# Autodesk Inventor assembly: assembly1
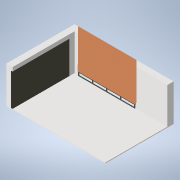
[picture p0: Inventor's stored thumbnail of the model, 180x180]
Saved by Autodesk Inventor 2021 (Build 250183000, 183)
## iProperties
Created: 2023-12-08
Part Number: assembly1
Document SubType Name: Assembly
Designer: assman
Author: assman
## Documents named in this file (5)
- D:\3DPrinting\3DModels\roco\assembly1.iam
- D:\3DPrinting\3DModels\roco\static.ipt
- D:\3DPrinting\3DModels\roco\structure.ipt
- D:\3DPrinting\3DModels\roco\zocalo_superior.ipt
- D:\3DPrinting\3DModels\roco\madera.ipt
## Components (6 placed, 4 different names)
1. static:1 — Mate:1, Mate:2, Mate:3
2. structure:1 — Mate:1, Mate:2, Mate:3, Rotational:1
3. zocalo_superior:1 — Rotational:1, Mate:4, Mate:5, Mate:6, Mate:8, Mate:9, Mate:11
4. madera:1 — Mate:4, Mate:5, Mate:7
5. madera:2 — Mate:6, Mate:7, Mate:8, Mate:10
6. madera:3 — Mate:9, Mate:10, Mate:11
## Relationships (12: Mate 11, RevoluteJoint 1)
- Mate:1 (270 mm): static:1 ↔ structure:1
- Mate:2: static:1 ↔ structure:1
- Mate:3: static:1 ↔ structure:1
- Rotational:1 [RevoluteJoint]: structure:1 ↔ zocalo_superior:1
- Mate:4: zocalo_superior:1 ↔ madera:1
- Mate:5: zocalo_superior:1 ↔ madera:1
- Mate:6: zocalo_superior:1 ↔ madera:2
- Mate:7: madera:1 ↔ madera:2
- Mate:8: zocalo_superior:1 ↔ madera:2
- Mate:9: zocalo_superior:1 ↔ madera:3
- Mate:10: madera:2 ↔ madera:3
- Mate:11: zocalo_superior:1 ↔ madera:3
